# Autodesk Inventor assembly: Drivetrain Motor Sprocket
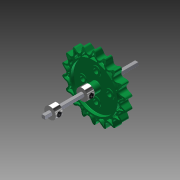
[picture p0: Inventor's stored thumbnail of the model, 180x180]
Saved by Autodesk Inventor 2012 (Build 160160000, 160)
## iProperties
Created: 2011-09-10
Part Number: Drivetrain Motor Sprocket
Document SubType Name: Assembly
Designer: Wade
Author: Wade
## Documents named in this file (5)
- C:\Users\Wade\Documents\1103 Robot - CAD Assembly\Drivetrain Motor Sprocket.iam
- C:\Users\Wade\Documents\1103 Robot - CAD Assembly\18 Tooth HS Sprocket.ipt
- C:\Users\Wade\Documents\1103 Robot - CAD Assembly\4 inch Shaft.ipt
- C:\Users\Wade\Documents\24C VEX CAD Files\Other Parts\Shaft Collar (with Set Screw Installed).ipt
- C:\Users\Wade\Documents\24C VEX CAD Files\Washers & Spacers\Washer, Delrin.ipt
## Components (5 placed, 4 different names)
1. 18 Tooth HS Sprocket:1 — Mate:1, Mate:2, Mate:3, Mate:4, Mate:5, Mate:6, Mate:7
2. 4 inch Shaft:1 — Flush:1, Mate:6, Mate:7, Flush:3, Flush:4, Flush:5
3. Shaft Collar (with Set Screw Installed):1 — Mate:1, Mate:4, Flush:4
4. Shaft Collar (with Set Screw Installed):2 — Mate:2, Flush:1, Flush:3
5. Washer, Delrin:1 — Mate:3, Mate:5, Flush:5
## Relationships (11: Mate 7, Flush 4)
- Mate:1: 18 Tooth HS Sprocket:1 ↔ Shaft Collar (with Set Screw Installed):1
- Mate:2: 18 Tooth HS Sprocket:1 ↔ Shaft Collar (with Set Screw Installed):2
- Mate:3: 18 Tooth HS Sprocket:1 ↔ Washer, Delrin:1
- Flush:1 (6.35 mm): 4 inch Shaft:1 ↔ Shaft Collar (with Set Screw Installed):2
- Mate:4: 18 Tooth HS Sprocket:1 ↔ Shaft Collar (with Set Screw Installed):1
- Mate:5: 18 Tooth HS Sprocket:1 ↔ Washer, Delrin:1
- Mate:6: 18 Tooth HS Sprocket:1 ↔ 4 inch Shaft:1
- Mate:7: 18 Tooth HS Sprocket:1 ↔ 4 inch Shaft:1
- Flush:3: 4 inch Shaft:1 ↔ Shaft Collar (with Set Screw Installed):2
- Flush:4: 4 inch Shaft:1 ↔ Shaft Collar (with Set Screw Installed):1
- Flush:5 (28.575 mm): 4 inch Shaft:1 ↔ Washer, Delrin:1
